# Autodesk Inventor assembly: 220LB-ASSY_MIR
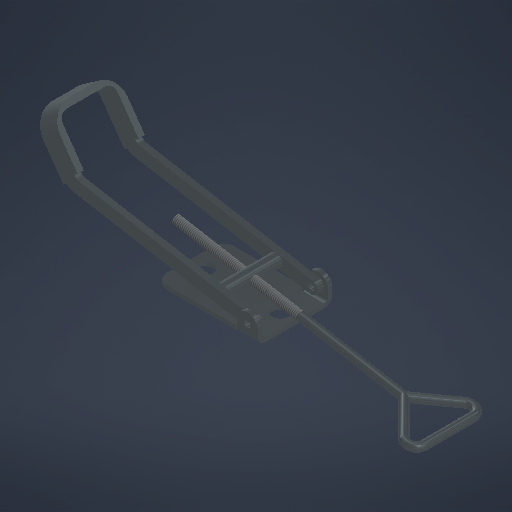
[picture p0: Inventor's stored thumbnail of the model, 512x512]
Saved by Autodesk Inventor 2025.3 (Build 293356030, 356C)
## iProperties
Created: 2025-08-31
Part Number: 220LB-ASSY_MIR
Document SubType Name: Assembly
Designer: K1NG
Author: lstk1ng
## Documents named in this file (4)
- C:\Users\lstk1ng\Documents\UPC\UPC-10\PROYECTO MECATRONICO 1\DISEÑO MECANICO\220LB LOCK\220LB-ASSY_MIR.iam
- C:\Users\lstk1ng\Documents\UPC\UPC-10\PROYECTO MECATRONICO 1\DISEÑO MECANICO\220LB LOCK\BODY-220LB_MIR.ipt
- C:\Users\lstk1ng\Documents\UPC\UPC-10\PROYECTO MECATRONICO 1\DISEÑO MECANICO\220LB LOCK\GRIPPER-220LB_MIR.ipt
- C:\Users\lstk1ng\Documents\UPC\UPC-10\PROYECTO MECATRONICO 1\DISEÑO MECANICO\220LB LOCK\PLATE-220_MIR.ipt
## Components (3 placed, 3 different names)
1. BODY-220LB_MIR:1 — Insert:1, Mate:1, Cylindrical:1
2. GRIPPER-220LB_MIR:1 — Cylindrical:1
3. PLATE-220_MIR:1 — Insert:1, Mate:1
## Relationships (3: Insert 1, Mate 1, CylindricalJoint 1)
- Insert:1: BODY-220LB_MIR:1 ↔ PLATE-220_MIR:1
- Mate:1: BODY-220LB_MIR:1 ↔ PLATE-220_MIR:1
- Cylindrical:1: BODY-220LB_MIR:1 ↔ GRIPPER-220LB_MIR:1
